# Autodesk Inventor assembly: Assembly new
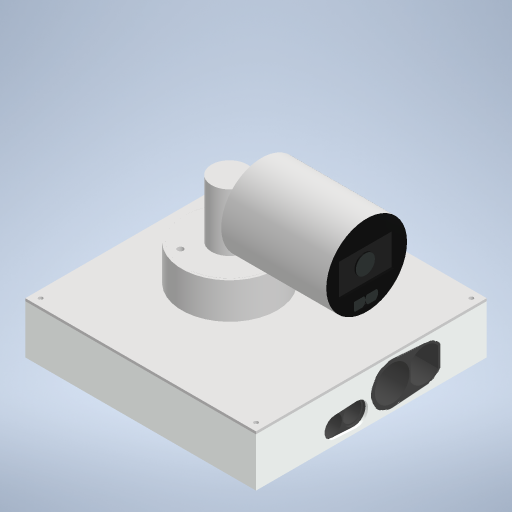
[picture p0: Inventor's stored thumbnail of the model, 512x512]
Saved by Autodesk Inventor 2024.3 (Build 283343000, 343)
## iProperties
Created: 2026-03-19
Part Number: Assembly new
Document SubType Name: Assembly
Designer: User
Author: User
## Documents named in this file (7)
- C:\Users\Pongpiched Rakshit\VisonLRF\3D_Models\Assembly.iam
- C:\Users\Pongpiched Rakshit\VisonLRF\3D_Models\Base plate.ipt
- C:\Users\Pongpiched Rakshit\VisonLRF\3D_Models\Top plate.ipt
- C:\Users\Pongpiched Rakshit\VisonLRF\3D_Models\3000m LRF.ipt
- C:\Users\Pongpiched Rakshit\VisonLRF\3D_Models\400m LRF.ipt
- C:\Users\Pongpiched Rakshit\VisonLRF\3D_Models\Camera.ipt
- C:\Users\Pongpiched Rakshit\VisonLRF\3D_Models\USB hub.ipt
## Components (6 placed, 6 different names)
1. Base plate:1 — Flush:2, Mate:1, Mate:2, Insert:1, Mate:3, Flush:3, Flush:4, Mate:4, Mate:5
2. Top plate:1 — Mate:3, Flush:3, Flush:4, Insert:2, Insert:3
3. 3000m LRF:1 — Flush:2
4. 400m LRF:1 — Mate:1, Mate:2, Insert:1
5. Camera:1 — Insert:2, Insert:3
6. USB hub:1 — Mate:4, Mate:5
## Relationships (11: Mate 5, Flush 3, Insert 3)
- Flush:2: Base plate:1 ↔ 3000m LRF:1
- Mate:1: Base plate:1 ↔ 400m LRF:1
- Mate:2: Base plate:1 ↔ 400m LRF:1
- Insert:1: Base plate:1 ↔ 400m LRF:1
- Mate:3: Base plate:1 ↔ Top plate:1
- Flush:3: Base plate:1 ↔ Top plate:1
- Flush:4: Base plate:1 ↔ Top plate:1
- Insert:2: Top plate:1 ↔ Camera:1
- Insert:3: Top plate:1 ↔ Camera:1
- Mate:4: Base plate:1 ↔ USB hub:1
- Mate:5: Base plate:1 ↔ USB hub:1
